# Autodesk Inventor assembly: Body
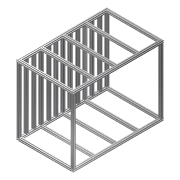
[picture p0: Inventor's stored thumbnail of the model, 180x180]
Saved by Autodesk Inventor 2019 (Build 230136000, 136)
## iProperties
Created: 2019-04-15
Part Number: Body
Material: 일반
Document SubType Name: Assembly
Designer: hinmo
Mass: 3292.36 g
Surface Area: 16544.1 cm^2
Volume: 1219.39 cm^3
Density: 2.7 g/cm^3
Author: hinmo
## Documents named in this file (4)
- C:\Users\hinmo\Documents\Inventor\Projects\2019_CapstoneDesign\Body.iam
- C:\Users\hinmo\Documents\Inventor\Projects\2019_CapstoneDesign\Propile_202070.ipt
- C:\Users\hinmo\Documents\Inventor\Projects\2019_CapstoneDesign\Propile_202050.ipt
- C:\Users\hinmo\Documents\Inventor\Projects\2019_CapstoneDesign\Propile_202040.ipt
## Components (29 placed, 3 different names)
1. Propile_202070:1 — 메이트:4, 메이트:5, 플러쉬:7, 플러쉬:8, 플러쉬:11, 플러쉬:12, 메이트:9, 메이트:10, 플러쉬:13, 플러쉬:14, 메이트:15, 플러쉬:28
2. Propile_202070:2 — 메이트:1, 플러쉬:1, 플러쉬:2, 메이트:3, 플러쉬:5, 플러쉬:6, 메이트:11, 플러쉬:21, 메이트:40, 메이트:41, 메이트:42, 플러쉬:39, 플러쉬:40, 플러쉬:41
3. Propile_202070:3 — 메이트:6, 플러쉬:9, 플러쉬:10, 메이트:7, 메이트:8, 플러쉬:15, 플러쉬:16, 메이트:12, 메이트:13, 메이트:14, 플러쉬:23, 플러쉬:24, 플러쉬:25, 메이트:16, 플러쉬:29, 메이트:17, 메이트:18, 메이트:19, 메이트:20, 메이트:21, 플러쉬:30, 플러쉬:31, 플러쉬:32, 플러쉬:33, 플러쉬:34, 메이트:22, 플러쉬:35
4. Propile_202070:4 — 메이트:2, 플러쉬:3, 플러쉬:4, 메이트:34, 메이트:35, 메이트:36, 플러쉬:36, 플러쉬:37, 플러쉬:38
5. Propile_202050:1 — 메이트:1, 메이트:2, 플러쉬:1, 플러쉬:2, 플러쉬:3, 플러쉬:4, 플러쉬:26, 플러쉬:27
6. Propile_202050:2 — 메이트:3, 플러쉬:5, 플러쉬:6, 플러쉬:22
7. Propile_202050:3 — 메이트:4, 메이트:6, 플러쉬:7, 플러쉬:8, 플러쉬:17, 플러쉬:18, 플러쉬:19, 플러쉬:20, 메이트:23, 메이트:32
8. Propile_202050:4 — 메이트:5, 플러쉬:9, 플러쉬:10, 플러쉬:11, 플러쉬:12, 메이트:27
9. Propile_202040:1 — 메이트:7, 플러쉬:15, 플러쉬:27, 메이트:39
10. Propile_202040:2 — 메이트:8, 플러쉬:16, 플러쉬:17, 플러쉬:19, 메이트:37, 메이트:38
11. Propile_202040:3 — 메이트:9, 플러쉬:14, 플러쉬:26, 메이트:44, 메이트:45
12. Propile_202040:4 — 메이트:10, 플러쉬:13, 플러쉬:18, 플러쉬:20, 메이트:11, 플러쉬:21, 플러쉬:22, 메이트:43
13. Propile_202050:5 — 메이트:12, 플러쉬:25, 메이트:27
14. Propile_202050:6 — 메이트:13, 플러쉬:24, 메이트:26
15. Propile_202050:7 — 메이트:14, 플러쉬:23, 메이트:25, 메이트:26, 메이트:28
16. Propile_202050:8 — 메이트:15, 플러쉬:28, 메이트:28
17. Propile_202050:9 — 메이트:16, 플러쉬:29, 메이트:29
18. Propile_202050:10 — 메이트:17, 플러쉬:30, 메이트:30, 메이트:33
19. Propile_202050:11 — 메이트:18, 플러쉬:31, 메이트:33
20. Propile_202050:12 — 메이트:19, 플러쉬:32, 메이트:24, 메이트:31
21. Propile_202050:13 — 메이트:20, 플러쉬:33, 메이트:31
22. Propile_202050:14 — 메이트:21, 플러쉬:34, 메이트:32
23. Propile_202050:15 — 메이트:22, 플러쉬:35, 메이트:23, 메이트:24, 메이트:25, 메이트:29, 메이트:30
24. Propile_202040:5 — 메이트:34, 플러쉬:36, 메이트:39
25. Propile_202040:6 — 메이트:35, 플러쉬:37, 메이트:37
26. Propile_202040:7 — 메이트:36, 플러쉬:38, 메이트:38
27. Propile_202040:8 — 메이트:40, 플러쉬:41, 메이트:44
28. Propile_202040:9 — 메이트:41, 플러쉬:40, 메이트:45
29. Propile_202040:10 — 메이트:42, 플러쉬:39, 메이트:43
## Relationships (86: Mate 45, Flush 41)
- 메이트:1 [Mate]: Propile_202070:2 ↔ Propile_202050:1
- 메이트:2 [Mate]: Propile_202070:4 ↔ Propile_202050:1
- 플러쉬:1 [Flush]: Propile_202070:2 ↔ Propile_202050:1
- 플러쉬:2 [Flush]: Propile_202070:2 ↔ Propile_202050:1
- 플러쉬:3 [Flush]: Propile_202070:4 ↔ Propile_202050:1
- 플러쉬:4 [Flush]: Propile_202070:4 ↔ Propile_202050:1
- 메이트:3 [Mate]: Propile_202070:2 ↔ Propile_202050:2
- 플러쉬:5 [Flush]: Propile_202070:2 ↔ Propile_202050:2
- 플러쉬:6 [Flush]: Propile_202070:2 ↔ Propile_202050:2
- 메이트:4 [Mate]: Propile_202070:1 ↔ Propile_202050:3
- 메이트:5 [Mate]: Propile_202070:1 ↔ Propile_202050:4
- 메이트:6 [Mate]: Propile_202070:3 ↔ Propile_202050:3
- 플러쉬:7 [Flush]: Propile_202070:1 ↔ Propile_202050:3
- 플러쉬:8 [Flush]: Propile_202070:1 ↔ Propile_202050:3
- 플러쉬:9 [Flush]: Propile_202070:3 ↔ Propile_202050:4
- 플러쉬:10 [Flush]: Propile_202070:3 ↔ Propile_202050:4
- 플러쉬:11 [Flush]: Propile_202070:1 ↔ Propile_202050:4
- 플러쉬:12 [Flush]: Propile_202070:1 ↔ Propile_202050:4
- 메이트:7 [Mate]: Propile_202070:3 ↔ Propile_202040:1
- 메이트:8 [Mate]: Propile_202070:3 ↔ Propile_202040:2
- 메이트:9 [Mate]: Propile_202070:1 ↔ Propile_202040:3
- 메이트:10 [Mate]: Propile_202070:1 ↔ Propile_202040:4
- 플러쉬:13 [Flush]: Propile_202070:1 ↔ Propile_202040:4
- 플러쉬:14 [Flush]: Propile_202070:1 ↔ Propile_202040:3
- 플러쉬:15 [Flush]: Propile_202070:3 ↔ Propile_202040:1
- 플러쉬:16 [Flush]: Propile_202070:3 ↔ Propile_202040:2
- 플러쉬:17 [Flush]: Propile_202050:3 ↔ Propile_202040:2
- 플러쉬:18 [Flush]: Propile_202050:3 ↔ Propile_202040:4
- 플러쉬:19 [Flush]: Propile_202050:3 ↔ Propile_202040:2
- 플러쉬:20 [Flush]: Propile_202050:3 ↔ Propile_202040:4
- 메이트:11 [Mate]: Propile_202070:2 ↔ Propile_202040:4
- 플러쉬:21 [Flush]: Propile_202070:2 ↔ Propile_202040:4
- 플러쉬:22 [Flush]: Propile_202050:2 ↔ Propile_202040:4
- 메이트:12 [Mate]: Propile_202070:3 ↔ Propile_202050:5
- 메이트:13 [Mate]: Propile_202070:3 ↔ Propile_202050:6
- 메이트:14 [Mate]: Propile_202070:3 ↔ Propile_202050:7
- 플러쉬:23 [Flush]: Propile_202070:3 ↔ Propile_202050:7
- 플러쉬:24 [Flush]: Propile_202070:3 ↔ Propile_202050:6
- 플러쉬:25 [Flush]: Propile_202070:3 ↔ Propile_202050:5
- 플러쉬:26 [Flush]: Propile_202050:1 ↔ Propile_202040:3
- 플러쉬:27 [Flush]: Propile_202050:1 ↔ Propile_202040:1
- 메이트:15 [Mate]: Propile_202070:1 ↔ Propile_202050:8
- 플러쉬:28 [Flush]: Propile_202070:1 ↔ Propile_202050:8
- 메이트:16 [Mate]: Propile_202070:3 ↔ Propile_202050:9
- 플러쉬:29 [Flush]: Propile_202070:3 ↔ Propile_202050:9
- 메이트:17 [Mate]: Propile_202070:3 ↔ Propile_202050:10
- 메이트:18 [Mate]: Propile_202070:3 ↔ Propile_202050:11
- 메이트:19 [Mate]: Propile_202070:3 ↔ Propile_202050:12
- 메이트:20 [Mate]: Propile_202070:3 ↔ Propile_202050:13
- 메이트:21 [Mate]: Propile_202070:3 ↔ Propile_202050:14
- 플러쉬:30 [Flush]: Propile_202070:3 ↔ Propile_202050:10
- 플러쉬:31 [Flush]: Propile_202070:3 ↔ Propile_202050:11
- 플러쉬:32 [Flush]: Propile_202070:3 ↔ Propile_202050:12
- 플러쉬:33 [Flush]: Propile_202070:3 ↔ Propile_202050:13
- 플러쉬:34 [Flush]: Propile_202070:3 ↔ Propile_202050:14
- 메이트:22 [Mate]: Propile_202070:3 ↔ Propile_202050:15
- 플러쉬:35 [Flush]: Propile_202070:3 ↔ Propile_202050:15
- 메이트:23 [Mate] (320 mm): Propile_202050:3 ↔ Propile_202050:15
- 메이트:24 [Mate] (150 mm): Propile_202050:12 ↔ Propile_202050:15
- 메이트:25 [Mate] (150 mm): Propile_202050:7 ↔ Propile_202050:15
- 메이트:26 [Mate] (35 mm): Propile_202050:6 ↔ Propile_202050:7
- 메이트:27 [Mate] (35 mm): Propile_202050:4 ↔ Propile_202050:5
- 메이트:28 [Mate] (35 mm): Propile_202050:7 ↔ Propile_202050:8
- 메이트:29 [Mate] (35 mm): Propile_202050:9 ↔ Propile_202050:15
- 메이트:30 [Mate] (35 mm): Propile_202050:10 ↔ Propile_202050:15
- 메이트:31 [Mate] (35 mm): Propile_202050:12 ↔ Propile_202050:13
- 메이트:32 [Mate] (35 mm): Propile_202050:3 ↔ Propile_202050:14
- 메이트:33 [Mate] (35 mm): Propile_202050:10 ↔ Propile_202050:11
- 메이트:34 [Mate]: Propile_202070:4 ↔ Propile_202040:5
- 메이트:35 [Mate]: Propile_202070:4 ↔ Propile_202040:6
- 메이트:36 [Mate]: Propile_202070:4 ↔ Propile_202040:7
- 플러쉬:36 [Flush]: Propile_202070:4 ↔ Propile_202040:5
- 플러쉬:37 [Flush]: Propile_202070:4 ↔ Propile_202040:6
- 플러쉬:38 [Flush]: Propile_202070:4 ↔ Propile_202040:7
- 메이트:37 [Mate] (320 mm): Propile_202040:2 ↔ Propile_202040:6
- 메이트:38 [Mate] (150 mm): Propile_202040:2 ↔ Propile_202040:7
- 메이트:39 [Mate] (150 mm): Propile_202040:1 ↔ Propile_202040:5
- 메이트:40 [Mate]: Propile_202070:2 ↔ Propile_202040:8
- 메이트:41 [Mate]: Propile_202070:2 ↔ Propile_202040:9
- 메이트:42 [Mate]: Propile_202070:2 ↔ Propile_202040:10
- 플러쉬:39 [Flush]: Propile_202070:2 ↔ Propile_202040:10
- 플러쉬:40 [Flush]: Propile_202070:2 ↔ Propile_202040:9
- 플러쉬:41 [Flush]: Propile_202070:2 ↔ Propile_202040:8
- 메이트:43 [Mate] (150 mm): Propile_202040:4 ↔ Propile_202040:10
- 메이트:44 [Mate] (150 mm): Propile_202040:3 ↔ Propile_202040:8
- 메이트:45 [Mate] (320 mm): Propile_202040:3 ↔ Propile_202040:9
